# Autodesk Inventor assembly: Ensamblaje
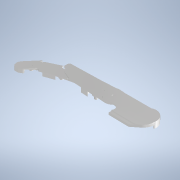
[picture p0: Inventor's stored thumbnail of the model, 180x180]
Saved by Autodesk Inventor 2022 (Build 260153000, 153)
## iProperties
Created: 2022-11-04
Part Number: Ensamblaje
Document SubType Name: Assembly
Designer: Mauricio Guerrero
Author: Mauricio Guerrero
## Documents named in this file (8)
- C:\Users\Griselda Hernandez\Documents\FIME\7mo Semestre\Biomecanica\PIA\Ensamblaje.iam
- C:\Users\Griselda Hernandez\Documents\FIME\7mo Semestre\Biomecanica\PIA\Pieza4.ipt
- C:\Users\Griselda Hernandez\Documents\FIME\7mo Semestre\Biomecanica\PIA\Pieza1.ipt
- C:\Users\Griselda Hernandez\Documents\FIME\7mo Semestre\Biomecanica\PIA\Pieza2.ipt
- C:\Users\Griselda Hernandez\Documents\FIME\7mo Semestre\Biomecanica\PIA\Pieza3.ipt
- C:\Users\Griselda Hernandez\Documents\FIME\7mo Semestre\Biomecanica\PIA\Pieza5.ipt
- C:\Users\Griselda Hernandez\Documents\FIME\7mo Semestre\Biomecanica\PIA\Pieza8.ipt
- C:\Users\Griselda Hernandez\Documents\FIME\7mo Semestre\Biomecanica\PIA\Pieza9.ipt
## Components (7 placed, 7 different names)
1. Pieza4:1 — Coincidencia:1, Coincidencia:2
2. Pieza1:1 — Coincidencia:1, Coincidencia:2, Coincidencia:3, Coincidencia:4, Coincidencia:14, Coincidencia:15, Coincidencia:19, Coincidencia:21, Coincidencia:24
3. Pieza2:1 — Coincidencia:3, Coincidencia:4, Coincidencia:5, Coincidencia:6, Coincidencia:23
4. Pieza3:1 — Coincidencia:5, Coincidencia:6, Coincidencia:20
5. Pieza5:1 — Coincidencia:14, Coincidencia:15, Coincidencia:22
6. Pieza9:2 — Coincidencia:19, Coincidencia:20, Coincidencia:21
7. Pieza8:2 — Coincidencia:22, Coincidencia:23, Coincidencia:24
## Relationships (14: Mate 14)
- Coincidencia:1 [Mate]: Pieza4:1 ↔ Pieza1:1
- Coincidencia:2 [Mate]: Pieza4:1 ↔ Pieza1:1
- Coincidencia:3 [Mate]: Pieza1:1 ↔ Pieza2:1
- Coincidencia:4 [Mate]: Pieza1:1 ↔ Pieza2:1
- Coincidencia:5 [Mate]: Pieza2:1 ↔ Pieza3:1
- Coincidencia:6 [Mate]: Pieza2:1 ↔ Pieza3:1
- Coincidencia:14 [Mate]: Pieza1:1 ↔ Pieza5:1
- Coincidencia:15 [Mate]: Pieza1:1 ↔ Pieza5:1
- Coincidencia:19 [Mate]: Pieza1:1 ↔ Pieza9:2
- Coincidencia:20 [Mate]: Pieza3:1 ↔ Pieza9:2
- Coincidencia:21 [Mate]: Pieza1:1 ↔ Pieza9:2
- Coincidencia:22 [Mate]: Pieza5:1 ↔ Pieza8:2
- Coincidencia:23 [Mate]: Pieza2:1 ↔ Pieza8:2
- Coincidencia:24 [Mate]: Pieza1:1 ↔ Pieza8:2
